# Autodesk Inventor assembly: LongerChain
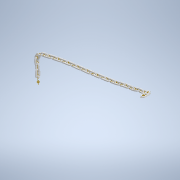
[picture p0: Inventor's stored thumbnail of the model, 180x180]
Saved by Autodesk Inventor 2021 (Build 250183000, 183)
## iProperties
Created: 2021-03-03
Part Number: LongerChain
Document SubType Name: Assembly
Designer: con_c_000
Author: con_c_000
## Documents named in this file (3)
- F:\PHRC CADD 2021\2021 Game Design Challenge\Anchor\LongerChain.iam
- F:\PHRC CADD 2021\2021 Game Design Challenge\Anchor\chainLink.ipt
- F:\PHRC CADD 2021\2021 Game Design Challenge\Anchor\chainLink2.ipt
## Components (29 placed, 2 different names)
1. chainLink:1
2. chainLink2:1
3. chainLink2:2
4. chainLink2:3
5. chainLink2:4
6. chainLink2:5
7. chainLink2:6
8. chainLink2:7
9. chainLink2:8
10. chainLink2:9
11. chainLink2:10
12. chainLink2:11
13. chainLink2:12
14. chainLink2:13
15. chainLink2:14
16. chainLink2:15
17. chainLink2:16
18. chainLink2:17
19. chainLink2:18
20. chainLink2:19
21. chainLink2:20
22. chainLink2:21
23. chainLink2:22
24. chainLink2:23
25. chainLink2:24
26. chainLink2:25
27. chainLink2:26
28. chainLink2:27
29. chainLink2:28
## Relationships (29: Composite 28, Flush 1)
- [Composite]: chainLink:1 ↔ chainLink2:1
- [Composite]: chainLink2:1 ↔ chainLink2:2
- [Composite]: chainLink2:2 ↔ chainLink2:3
- [Composite]: chainLink2:3 ↔ chainLink2:4
- [Composite]: chainLink2:4 ↔ chainLink2:5
- [Composite]: chainLink2:5 ↔ chainLink2:6
- [Composite]: chainLink2:6 ↔ chainLink2:7
- [Composite]: chainLink2:7 ↔ chainLink2:8
- [Composite]: chainLink2:8 ↔ chainLink2:9
- [Composite]: chainLink2:9 ↔ chainLink2:10
- [Composite]: chainLink2:10 ↔ chainLink2:11
- [Composite]: chainLink2:11 ↔ chainLink2:12
- [Composite]: chainLink2:12 ↔ chainLink2:13
- [Composite]: chainLink2:13 ↔ chainLink2:14
- [Composite]: chainLink2:14 ↔ chainLink2:15
- [Composite]: chainLink2:15 ↔ chainLink2:16
- [Composite]: chainLink2:16 ↔ chainLink2:17
- [Composite]: chainLink2:17 ↔ chainLink2:18
- [Composite]: chainLink2:18 ↔ chainLink2:19
- [Composite]: chainLink2:19 ↔ chainLink2:20
- [Composite]: chainLink2:20 ↔ chainLink2:21
- [Composite]: chainLink2:21 ↔ chainLink2:22
- [Composite]: chainLink2:22 ↔ chainLink2:23
- [Composite]: chainLink2:23 ↔ chainLink2:24
- [Composite]: chainLink2:24 ↔ chainLink2:25
- [Composite]: chainLink2:25 ↔ chainLink2:26
- [Composite]: chainLink2:26 ↔ chainLink2:27
- [Composite]: chainLink2:27 ↔ chainLink2:28
- Flush:1 (-254 mm)
